# Autodesk Inventor assembly: Assembly1
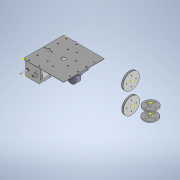
[picture p0: Inventor's stored thumbnail of the model, 180x180]
Saved by Autodesk Inventor 2021.3 (Build 253353000, 353)
## iProperties
Created: 2021-10-16
Part Number: Assembly1
Document SubType Name: Assembly
Designer: gilte
Author: gilte
## Documents named in this file (15)
- C:\Users\gilte\Documents\Inventor\kadai3\Assembly1.iam
- C:\Users\gilte\Desktop\設計制作論1\RD002_フレーム.ipt
- C:\Users\gilte\Desktop\設計制作論1\RD004_スペーサ.ipt
- C:\Users\gilte\Desktop\設計制作論1\RD003_キャスタ420G-R32.ipt
- C:\Users\gilte\Desktop\設計制作論1\RD005_ペンホルダ.ipt
- C:\Users\gilte\Desktop\設計制作論1\RD006_ギヤボックス左.ipt
- C:\Users\gilte\Desktop\設計制作論1\RD007_ギヤボックス右.ipt
- C:\Users\gilte\Documents\Inventor\kadai3\RD008_モータ(DMN29).ipt
- C:\Users\gilte\Desktop\設計制作論1\RD009_ギアDS0.5-12.ipt
- C:\Users\gilte\Desktop\設計制作論1\RD014_ストッパ.ipt
- C:\Users\gilte\Desktop\設計制作論1\RD015_シャフト.ipt
- C:\Users\gilte\Desktop\設計制作論1\RD019_ブッシュ80F-0305改.ipt
- C:\Users\gilte\Documents\Inventor\kadai3\RD020_ワッシャ.ipt
- C:\Users\gilte\Desktop\設計制作論1\RD012_ホイール.ipt
- C:\Users\gilte\Desktop\設計制作論1\RD010_ギアDS0.5-80.ipt
## Components (24 placed, 14 different names)
1. RD002_フレーム:1 — 挿入:1, 挿入:2, 挿入:4, 挿入:5, 挿入:6, 挿入:7, 挿入:8, 挿入:9, 挿入:10
2. RD004_スペーサ:1 — 挿入:1, 挿入:2, 挿入:3, 挿入:4
3. RD003_キャスタ420G-R32:1 — 挿入:3
4. RD005_ペンホルダ:1 — 挿入:5, 挿入:6
5. RD006_ギヤボックス左:1 — 挿入:7, 挿入:8, 挿入:13, 挿入:14, 挿入:17, 挿入:21
6. RD007_ギヤボックス右:1 — 挿入:9, 挿入:10, 挿入:11, 挿入:12, 挿入:18, 挿入:22
7. RD008_モータ(DMN29):1 — 挿入:13, 挿入:14, 挿入:16
8. RD008_モータ(DMN29):2 — 挿入:11, 挿入:12, 挿入:15
9. RD009_ギアDS0.5-12:1 — 挿入:16
10. RD009_ギアDS0.5-12:2 — 挿入:15
11. RD014_ストッパ:1 — 挿入:18, 挿入:20
12. RD014_ストッパ:2 — 挿入:17, 挿入:19
13. RD014_ストッパ:3
14. RD014_ストッパ:4
15. RD015_シャフト:1 — 挿入:19
16. RD015_シャフト:2 — 挿入:20
17. RD019_ブッシュ80F-0305改:1 — 挿入:22, 挿入:23
18. RD019_ブッシュ80F-0305改:2 — 挿入:21, 挿入:24
19. RD020_ワッシャ:1 — 挿入:24
20. RD020_ワッシャ:2 — 挿入:23
21. RD012_ホイール:1
22. RD012_ホイール:2
23. RD010_ギアDS0.5-80:1
24. RD010_ギアDS0.5-80:2
## Relationships (24: Insert 24)
- 挿入:1 [Insert]: RD002_フレーム:1 ↔ RD004_スペーサ:1
- 挿入:2 [Insert]: RD002_フレーム:1 ↔ RD004_スペーサ:1
- 挿入:3 [Insert]: RD004_スペーサ:1 ↔ RD003_キャスタ420G-R32:1
- 挿入:4 [Insert]: RD002_フレーム:1 ↔ RD004_スペーサ:1
- 挿入:5 [Insert]: RD002_フレーム:1 ↔ RD005_ペンホルダ:1
- 挿入:6 [Insert]: RD002_フレーム:1 ↔ RD005_ペンホルダ:1
- 挿入:7 [Insert]: RD002_フレーム:1 ↔ RD006_ギヤボックス左:1
- 挿入:8 [Insert]: RD002_フレーム:1 ↔ RD006_ギヤボックス左:1
- 挿入:9 [Insert]: RD002_フレーム:1 ↔ RD007_ギヤボックス右:1
- 挿入:10 [Insert]: RD002_フレーム:1 ↔ RD007_ギヤボックス右:1
- 挿入:11 [Insert]: RD007_ギヤボックス右:1 ↔ RD008_モータ(DMN29):2
- 挿入:12 [Insert]: RD007_ギヤボックス右:1 ↔ RD008_モータ(DMN29):2
- 挿入:13 [Insert]: RD006_ギヤボックス左:1 ↔ RD008_モータ(DMN29):1
- 挿入:14 [Insert]: RD006_ギヤボックス左:1 ↔ RD008_モータ(DMN29):1
- 挿入:15 [Insert]: RD008_モータ(DMN29):2 ↔ RD009_ギアDS0.5-12:2
- 挿入:16 [Insert]: RD008_モータ(DMN29):1 ↔ RD009_ギアDS0.5-12:1
- 挿入:17 [Insert]: RD006_ギヤボックス左:1 ↔ RD014_ストッパ:2
- 挿入:18 [Insert]: RD007_ギヤボックス右:1 ↔ RD014_ストッパ:1
- 挿入:19 [Insert]: RD014_ストッパ:2 ↔ RD015_シャフト:1
- 挿入:20 [Insert]: RD014_ストッパ:1 ↔ RD015_シャフト:2
- 挿入:21 [Insert]: RD006_ギヤボックス左:1 ↔ RD019_ブッシュ80F-0305改:2
- 挿入:22 [Insert]: RD007_ギヤボックス右:1 ↔ RD019_ブッシュ80F-0305改:1
- 挿入:23 [Insert]: RD019_ブッシュ80F-0305改:1 ↔ RD020_ワッシャ:2
- 挿入:24 [Insert]: RD019_ブッシュ80F-0305改:2 ↔ RD020_ワッシャ:1
